# Autodesk Inventor assembly: foot type 1
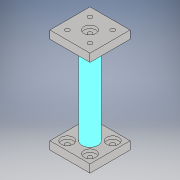
[picture p0: Inventor's stored thumbnail of the model, 180x180]
Saved by Autodesk Inventor 2018 (Build 220112000, 112)
## iProperties
Created: 2018-10-16
Part Number: foot type 1
Document SubType Name: Assembly
Designer: freyja
Author: freyja
## Documents named in this file (3)
- C:\Users\freyja\Documents\Cryorefrigerator\CAD\foot type 1.iam
- C:\Users\freyja\Documents\Cryorefrigerator\CAD\feet type 1 part 1.ipt
- C:\Users\freyja\Documents\Cryorefrigerator\CAD\feet type 1 part 2.ipt
## Components (3 placed, 2 different names)
1. feet type 1 part 1:1 — Mate:1, Mate:2
2. feet type 1 part 2:1 — Mate:1, Mate:2, Mate:3, Mate:4
3. feet type 1 part 1:2 — Mate:3, Mate:4
## Relationships (4: Mate 4)
- Mate:1: feet type 1 part 1:1 ↔ feet type 1 part 2:1
- Mate:2: feet type 1 part 1:1 ↔ feet type 1 part 2:1
- Mate:3: feet type 1 part 2:1 ↔ feet type 1 part 1:2
- Mate:4: feet type 1 part 2:1 ↔ feet type 1 part 1:2
